# Autodesk Inventor assembly: 73. Шестерня третьей передачи в сборе
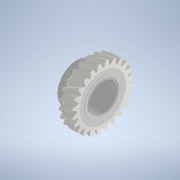
[picture p0: Inventor's stored thumbnail of the model, 180x180]
Saved by Autodesk Inventor 2021 (Build 250183000, 183)
## iProperties
Created: 2021-04-06
Part Number: 73. Шестерня третьей передачи в сборе
Document SubType Name: Assembly
Designer: Данил
Author: Данил
## Documents named in this file (3)
- C:\Users\Данил\Desktop\Коробка передач\Детали\73. Шестерня третьей передачи в сборе.iam
- C:\Users\Данил\Desktop\Коробка передач\Детали\73. Шестерня третьей передачи.iam
- C:\Users\Данил\Desktop\Коробка передач\Детали\75. Втулка шестерни третьей передачи.ipt
## Components (2 placed, 2 different names)
1. 73. Шестерня третьей передачи:1 [sub-assembly] — Совмещение:1, Заподлицо:1
2. 75. Втулка шестерни третьей передачи:1 — Совмещение:1, Заподлицо:1
## Relationships (2: Mate 1, Flush 1)
- Совмещение:1 [Mate]: 73. Шестерня третьей передачи:1 ↔ 75. Втулка шестерни третьей передачи:1
- Заподлицо:1 [Flush]: 73. Шестерня третьей передачи:1 ↔ 75. Втулка шестерни третьей передачи:1
